# Autodesk Inventor assembly: bumper test
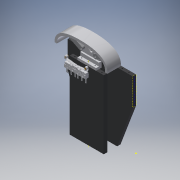
[picture p0: Inventor's stored thumbnail of the model, 180x180]
Saved by Autodesk Inventor 2016 (Build 200138000, 138)
## iProperties
Created: 2015-09-30
Part Number: bumper test
Document SubType Name: Assembly
Designer: Jesse Stevenson
Author: Jesse Stevenson
## Documents named in this file (7)
- C:\Users\Jesse Stevenson\Desktop\E-121-Design\bumper test.iam
- C:\Users\Jesse Stevenson\Desktop\E-121-Design\top.ipt
- C:\Users\Jesse Stevenson\Desktop\E-121-Design\bottom.ipt
- C:\Users\Jesse Stevenson\Desktop\E-121-Design\Microswitch_-_Omron_D2SW-P2L2T.iam
- C:\Users\Jesse Stevenson\Desktop\E-121-Design\bumper lever support.ipt
- C:\Users\Jesse Stevenson\Desktop\E-121-Design\lever2.ipt
- C:\Users\Jesse Stevenson\Desktop\E-121-Design\bumper.ipt
## Components (8 placed, 6 different names)
1. top:1 — Flush:1, Mate:1, Mate:2
2. bottom:1 — Flush:1, Mate:1, Mate:3, Mate:5, Mate:6, Flush:3, Flush:4
3. Microswitch_-_Omron_D2SW-P2L2T:1 [sub-assembly] — Mate:5, Mate:7, Flush:2
4. Microswitch_-_Omron_D2SW-P2L2T:2 [sub-assembly] — Mate:6, Mate:7, Flush:2
5. bumper lever support:1 — Flush:3, Flush:4, Mate:8, Mate:10, Mate:12, Mate:14
6. bumper:1 — Mate:13
7. lever2:1 — Mate:8, Mate:14
8. lever2:2 — Mate:10, Mate:12, Mate:13
## Relationships (16: Mate 12, Flush 4)
- Flush:1: top:1 ↔ bottom:1
- Mate:1 (18.923 mm): top:1 ↔ bottom:1
- Mate:2: top:1
- Mate:3: bottom:1
- Mate:4 (25.273 mm)
- Mate:5 (12.7 mm): bottom:1 ↔ Microswitch_-_Omron_D2SW-P2L2T:1
- Mate:6 (12.7 mm): bottom:1 ↔ Microswitch_-_Omron_D2SW-P2L2T:2
- Mate:7: Microswitch_-_Omron_D2SW-P2L2T:1 ↔ Microswitch_-_Omron_D2SW-P2L2T:2
- Flush:2: Microswitch_-_Omron_D2SW-P2L2T:1 ↔ Microswitch_-_Omron_D2SW-P2L2T:2
- Flush:3: bottom:1 ↔ bumper lever support:1
- Flush:4: bottom:1 ↔ bumper lever support:1
- Mate:8: bumper lever support:1 ↔ lever2:1
- Mate:10: bumper lever support:1 ↔ lever2:2
- Mate:12: bumper lever support:1 ↔ lever2:2
- Mate:13: bumper:1 ↔ lever2:2
- Mate:14: bumper lever support:1 ↔ lever2:1
